# Autodesk Inventor assembly: Main Assembly Spider Crab
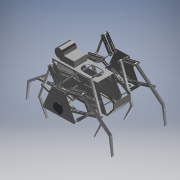
[picture p0: Inventor's stored thumbnail of the model, 180x180]
Saved by Autodesk Inventor 2019 (Build 230136000, 136)
## iProperties
Created: 2019-08-25
Part Number: Main Assembly Spider Crab
Document SubType Name: Assembly
Designer: DIBYOJYOTI
Mass: 4559.56 g
Surface Area: 6924.71 cm^2
Volume: 716.614 cm^3
Density: 6.36265 g/cm^3
Author: DIBYOJYOTI
## Documents named in this file (5)
- D:\TITO\Autocad\Main Assembly Spider Crab.iam
- D:\TITO\Autocad\Leg Pair Assembly Spider Crab.iam
- D:\TITO\Autocad\Flywheel.ipt
- D:\TITO\Autocad\Cabin Assembly.iam
- D:\TITO\Autocad\Crank Joint Pin extended Spider Crab.ipt
## Components (5 placed, 4 different names)
1. Leg Pair Assembly Spider Crab:1 [sub-assembly] — Insert:1, Insert:2, Insert:3, Insert:4, Rigid:2
2. Leg Pair Assembly Spider Crab:2 [sub-assembly] — Insert:5, Insert:6, Insert:7, Insert:8, Rigid:1, Rigid:3, Angle:1
3. Cabin Assembly:1 [sub-assembly] — Insert:1, Insert:2, Insert:3, Insert:4, Insert:5, Insert:6, Insert:7, Insert:8
4. Flywheel:1 — Rigid:3, Angle:1
5. Crank Joint Pin extended Spider Crab:1 — Rigid:1, Rigid:2
## Relationships (12: Insert 8, WeldJoint 3, Angle 1)
- Insert:1: Leg Pair Assembly Spider Crab:1 ↔ Cabin Assembly:1
- Insert:2: Leg Pair Assembly Spider Crab:1 ↔ Cabin Assembly:1
- Insert:3: Leg Pair Assembly Spider Crab:1 ↔ Cabin Assembly:1
- Insert:4: Leg Pair Assembly Spider Crab:1 ↔ Cabin Assembly:1
- Insert:5: Leg Pair Assembly Spider Crab:2 ↔ Cabin Assembly:1
- Insert:6: Leg Pair Assembly Spider Crab:2 ↔ Cabin Assembly:1
- Insert:7: Leg Pair Assembly Spider Crab:2 ↔ Cabin Assembly:1
- Insert:8: Leg Pair Assembly Spider Crab:2 ↔ Cabin Assembly:1
- Rigid:1 [WeldJoint]: Leg Pair Assembly Spider Crab:2 ↔ Crank Joint Pin extended Spider Crab:1
- Rigid:2 [WeldJoint]: Leg Pair Assembly Spider Crab:1 ↔ Crank Joint Pin extended Spider Crab:1
- Rigid:3 [WeldJoint]: Leg Pair Assembly Spider Crab:2 ↔ Flywheel:1
- Angle:1 (-1440 deg): Leg Pair Assembly Spider Crab:2 ↔ Flywheel:1
